# Autodesk Inventor assembly: Zespół1
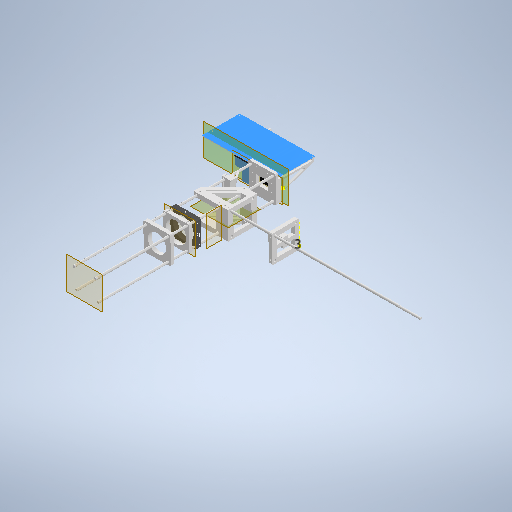
[picture p0: Inventor's stored thumbnail of the model, 512x512]
Saved by Autodesk Inventor 2025.1 (Build 291241000, 241)
## iProperties
Created: 2024-10-25
Part Number: Zespół1
Document SubType Name: Assembly
Designer: PC
Author: PC
## Documents named in this file (13)
- C:\Users\PC\Desktop\fotolito_czesci\nowe\main.iam
- C:\Users\PC\Desktop\fotolito_czesci\nowe\plyta_dmd.iam
- dmd_assembly.iam
- C:\Users\PC\Desktop\fotolito_czesci\rod.ipt
- C:\Users\PC\Desktop\fotolito_czesci\LCP09-Solidworks.ipt
- C:\Users\PC\Desktop\fotolito_czesci\nowe\wyliczenia.ipt
- C:\Users\PC\Desktop\fotolito_czesci\nowe\6_2xclamp_back.ipt
- C:\Users\PC\Desktop\fotolito_czesci\nowe\6_2xclamp_main.ipt
- C:\Users\PC\Desktop\fotolito_czesci\nowe\wzmocnienie.ipt
- C:\Users\PC\Desktop\fotolito_czesci\nowe\genera_ mount.ipt
- C:\Users\PC\Desktop\fotolito_czesci\nowe\mst.ipt
- C:\Users\PC\Desktop\fotolito_czesci\nowe\beamsplitter.ipt
- C:\Users\PC\Desktop\fotolito_czesci\nowe\camera_60mm.ipt
## Components (16 placed, 11 different names)
1. dmd_assembly:1 [sub-assembly] — Zestawiające:2, Zestawiające:3, Zestawiające:4, Zestawiające:5, Zestawiające:6, Równoległe:2, Kątowe:1, Zestawiające:8, Zestawiające:9, Zestawiające:12, Zestawiające:14, Zestawiające:16, Zestawiające:19, Zestawiające:21, Równoległe:3, Równoległe:6
2. rod:3 — Zestawiające:3, Zestawiające:5, Zestawiające:41, Zestawiające:43, Symetria:1
3. rod:4 — Zestawiające:4, Równoległe:2, Symetria:1, Zestawiające:44
4. rod:2 — Zestawiające:2, Zestawiające:6, Zestawiające:10, Zestawiające:23, Zestawiające:25, Zestawiające:45
5. LCP09-Solidworks:1 — Kątowe:1, Zestawiające:10
6. wyliczenia:1 — Zestawiające:8, Zestawiające:9, Zestawiające:11, Kątowe:2, Kątowe:3, Zestawiające:13, Kątowe:4, Kątowe:5, Zestawiające:15, Kątowe:6, Kątowe:7, Zestawiające:17, Kątowe:8, Zestawiające:18, Kątowe:9, Kątowe:10, Zestawiające:26, Zestawiające:27, Równoległe:5
7. rod:5 — Zestawiające:21, Równoległe:3, Zestawiające:22, Zestawiające:24, Zestawiające:40, Zestawiające:42
8. 6_2xclamp_back:1 — Zestawiające:24, Zestawiające:25, Równoległe:4
9. 6_2xclamp_main:1 — Zestawiające:22, Zestawiające:23, Równoległe:4, Zestawiające:26, Zestawiające:27, Równoległe:5
10. wzmocnienie:1 — Równoległe:7, Równoległe:9
11. rod:6 — Równoległe:12, Zestawiające:46, Zestawiające:48
12. rod:7 — Równoległe:12, Zestawiające:47
13. genera_ mount:1 — Zestawiające:40, Zestawiające:41
14. mst:1 — Zestawiające:42, Zestawiające:43
15. beamsplitter:1 — Zestawiające:44, Zestawiające:45, Zestawiające:46, Zestawiające:47
16. camera_60mm:1 — Zestawiające:48
## Relationships (52: Mate 33, Angle 10, Flush 8, Symmetry 1)
- Zestawiające:2 [Mate]: dmd_assembly:1 ↔ rod:2
- Zestawiające:3 [Mate]: dmd_assembly:1 ↔ rod:3
- Zestawiające:4 [Mate]: dmd_assembly:1 ↔ rod:4
- Zestawiające:5 [Mate]: dmd_assembly:1 ↔ rod:3
- Zestawiające:6 [Mate]: dmd_assembly:1 ↔ rod:2
- Równoległe:2 [Flush]: dmd_assembly:1 ↔ rod:4
- Kątowe:1 [Angle] (0 deg): dmd_assembly:1 ↔ LCP09-Solidworks:1
- Zestawiające:8 [Mate]: dmd_assembly:1 ↔ wyliczenia:1
- Zestawiające:9 [Mate]: dmd_assembly:1 ↔ wyliczenia:1
- Zestawiające:10 [Mate]: rod:2 ↔ LCP09-Solidworks:1
- Zestawiające:11 [Mate]: wyliczenia:1
- Kątowe:2 [Angle] (0 deg): wyliczenia:1
- Zestawiające:12 [Mate]: dmd_assembly:1
- Kątowe:3 [Angle] (0 deg): wyliczenia:1
- Zestawiające:13 [Mate]: wyliczenia:1
- Kątowe:4 [Angle] (0 deg): wyliczenia:1
- Zestawiające:14 [Mate]: dmd_assembly:1
- Kątowe:5 [Angle] (0 deg): wyliczenia:1
- Zestawiające:15 [Mate]: wyliczenia:1
- Kątowe:6 [Angle] (0 deg): wyliczenia:1
- Zestawiające:16 [Mate]: dmd_assembly:1
- Kątowe:7 [Angle] (0 deg): wyliczenia:1
- Zestawiające:17 [Mate]: wyliczenia:1
- Kątowe:8 [Angle] (0 deg): wyliczenia:1
- Zestawiające:18 [Mate]: wyliczenia:1
- Kątowe:9 [Angle] (0 deg): wyliczenia:1
- Zestawiające:19 [Mate]: dmd_assembly:1
- Kątowe:10 [Angle] (0 deg): wyliczenia:1
- Zestawiające:21 [Mate]: dmd_assembly:1 ↔ rod:5
- Równoległe:3 [Flush]: dmd_assembly:1 ↔ rod:5
- Zestawiające:22 [Mate]: rod:5 ↔ 6_2xclamp_main:1
- Zestawiające:23 [Mate]: rod:2 ↔ 6_2xclamp_main:1
- Zestawiające:24 [Mate]: rod:5 ↔ 6_2xclamp_back:1
- Zestawiające:25 [Mate]: rod:2 ↔ 6_2xclamp_back:1
- Równoległe:4 [Flush]: 6_2xclamp_back:1 ↔ 6_2xclamp_main:1
- Zestawiające:26 [Mate]: wyliczenia:1 ↔ 6_2xclamp_main:1
- Zestawiające:27 [Mate]: wyliczenia:1 ↔ 6_2xclamp_main:1
- Równoległe:5 [Flush]: wyliczenia:1 ↔ 6_2xclamp_main:1
- Równoległe:6 [Flush] (7.5 mm): dmd_assembly:1
- Równoległe:7 [Flush]: wzmocnienie:1
- Równoległe:9 [Flush]: wzmocnienie:1
- Równoległe:12 [Flush]: rod:6 ↔ rod:7
- Zestawiające:40 [Mate]: rod:5 ↔ genera_ mount:1
- Zestawiające:41 [Mate]: rod:3 ↔ genera_ mount:1
- Zestawiające:42 [Mate]: rod:5 ↔ mst:1
- Zestawiające:43 [Mate]: rod:3 ↔ mst:1
- Symetria:1 [Symmetry]: rod:3 ↔ rod:4
- Zestawiające:44 [Mate]: rod:4 ↔ beamsplitter:1
- Zestawiające:45 [Mate]: rod:2 ↔ beamsplitter:1
- Zestawiające:46 [Mate]: rod:6 ↔ beamsplitter:1
- Zestawiające:47 [Mate]: rod:7 ↔ beamsplitter:1
- Zestawiające:48 [Mate]: rod:6 ↔ camera_60mm:1
